# Autodesk Inventor assembly: Hanging Cupboard for Hood
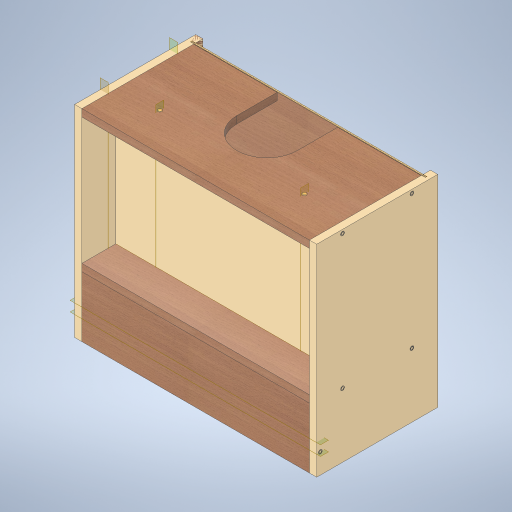
[picture p0: Inventor's stored thumbnail of the model, 512x512]
Saved by Autodesk Inventor 2024 (Build 280153000, 153)
## iProperties
RuleStatus: InUse
Created: 2017-01-20
Part Number: Hanging Cupboard for Hood
Document SubType Name: Assembly
Designer: SvetlanaB
Author: SvetlanaB
## Documents named in this file (12)
- C:\W4INV 2024 Design\iBOX LIBRARY\Kitchen\Wall Cabinets\Cupboard for Hood\Cupboard for Hood.iam
- C:\W4INV 2024 Design\iBOX LIBRARY\Kitchen\Wall Cabinets\Cupboard for Hood\Top panel.ipt
- C:\W4INV 2024 Design\iBOX LIBRARY\Kitchen\Wall Cabinets\Cupboard for Hood\Right panel.ipt
- C:\W4INV 2024 Design\iBOX LIBRARY\Kitchen\Wall Cabinets\Cupboard for Hood\Left panel.ipt
- C:\W4INV 2024 Design\iBOX LIBRARY\Kitchen\Wall Cabinets\Cupboard for Hood\Top panel2.ipt
- C:\W4INV 2024 Design\iBOX LIBRARY\Kitchen\Wall Cabinets\Cupboard for Hood\Bottom panel.ipt
- C:\W4INV 2024 Design\iBOX LIBRARY\Kitchen\Wall Cabinets\Cupboard for Hood\Back panel_1.ipt
- C:\W4INV 2024 Design\_LIBRARY\Fixed joints\Confirmat\CONFIRMAT\Confirmat L50 NB T18 PB T 18.ipt
- C:\W4INV 2024 Design\iBOX LIBRARY\Kitchen\Wall Cabinets\Cupboard for Hood\Hood cupboard concept.ipt
- C:\W4INV 2024 Design\iBOX LIBRARY\Kitchen\Wall Cabinets\Cupboard for Hood\Vertical partition.ipt
- C:\W4INV 2024 Design\_LIBRARY\Fixed joints\Confirmat\CONFIRMAT\Confirmat L50 & Cap D10 NB T18 PB T 18.ipt
- C:\W4INV 2023 Design\LIBRARY\Fixed joints\Confirmat\CONFIRMAT.ipt
## Components (22 placed, 10 different names)
1. @Skeleton
2. Top panel:1 — Pillar Board Side Plane:2, Pillar Board Side Plane:4, Pillar Board Side Plane:5, Pillar Board Side Plane:7, Nestled Board Plane:12, Nestled Board Plane:14, Flush:22
3. Right panel:1 — Nestled Board Plane:1, Nestled Board Plane:2, Nestled Board Plane:3, Nestled Board Plane:4, Nestled Board Plane:9
4. Left panel:1 — Flush:1, Flush:2, Nestled Board Plane:5, Nestled Board Plane:6, Nestled Board Plane:7, Nestled Board Plane:8, Nestled Board Plane:10, Mate:29, Mate:30
5. Top panel2:1 — Pillar Board Side Plane:1, Pillar Board Side Plane:3, Pillar Board Side Plane:6, Pillar Board Side Plane:8, Nestled Board Plane:11, Nestled Board Plane:13
6. Bottom panel:1 — Flush:5, Pillar Board Side Plane:9, Pillar Board Side Plane:10
7. Back panel_1:1 — Mate:29, Flush:22, Mate:30
8. Confirmat L50 NB T18 PB T 18:1 — Axis Plane:1, Pillar Board Side Plane:1, Nestled Board Plane:1
9. Confirmat L50 NB T18 PB T 18:2 — Axis Plane:2, Pillar Board Side Plane:2, Nestled Board Plane:2
10. Confirmat L50 NB T18 PB T 18:3 — Axis Plane:3, Pillar Board Side Plane:3, Nestled Board Plane:3
11. Confirmat L50 NB T18 PB T 18:4 — Axis Plane:4, Pillar Board Side Plane:4, Nestled Board Plane:4
12. Confirmat L50 NB T18 PB T 18:5 — Axis Plane:5, Pillar Board Side Plane:5, Nestled Board Plane:5
13. Confirmat L50 NB T18 PB T 18:6 — Axis Plane:6, Pillar Board Side Plane:6, Nestled Board Plane:6
14. Confirmat L50 NB T18 PB T 18:7 — Axis Plane:7, Pillar Board Side Plane:7, Nestled Board Plane:7
15. Confirmat L50 NB T18 PB T 18:8 — Axis Plane:8, Pillar Board Side Plane:8, Nestled Board Plane:8
16. Confirmat L50 NB T18 PB T 18:9 — Nestled Board Plane:9, Pillar Board Side Plane:9, Axis Plane:9
17. Confirmat L50 NB T18 PB T 18:10 — Nestled Board Plane:10, Pillar Board Side Plane:10, Axis Plane:10
18. Vertical partition:1 — Flush:16, Flush:17, Pillar Board Side Plane:11, Pillar Board Side Plane:12, Pillar Board Side Plane:13, Pillar Board Side Plane:14
19. Confirmat L50 & Cap D10 NB T18 PB T 18:11 — Axis Plane:11, Nestled Board Plane:11, Pillar Board Side Plane:11
20. Confirmat L50 & Cap D10 NB T18 PB T 18:12 — Axis Plane:12, Nestled Board Plane:12, Pillar Board Side Plane:12
21. Confirmat L50 & Cap D10 NB T18 PB T 18:13 — Axis Plane:13, Nestled Board Plane:13, Pillar Board Side Plane:13
22. Confirmat L50 & Cap D10 NB T18 PB T 18:14 — Axis Plane:14, Nestled Board Plane:14, Pillar Board Side Plane:14
## Relationships (50: Mate 30, Flush 20)
- Flush:1 (-64 mm): Left panel:1
- Flush:2 (-64 mm): Left panel:1
- Flush:5 (-50 mm): Bottom panel:1
- Axis Plane:1 [Mate]: Confirmat L50 NB T18 PB T 18:1
- Pillar Board Side Plane:1 [Mate] (-9 mm): Top panel2:1 ↔ Confirmat L50 NB T18 PB T 18:1
- Nestled Board Plane:1 [Flush]: Right panel:1 ↔ Confirmat L50 NB T18 PB T 18:1
- Axis Plane:2 [Mate]: Confirmat L50 NB T18 PB T 18:2
- Pillar Board Side Plane:2 [Mate] (-9 mm): Top panel:1 ↔ Confirmat L50 NB T18 PB T 18:2
- Nestled Board Plane:2 [Flush]: Right panel:1 ↔ Confirmat L50 NB T18 PB T 18:2
- Axis Plane:3 [Mate]: Confirmat L50 NB T18 PB T 18:3
- Pillar Board Side Plane:3 [Mate] (-9 mm): Top panel2:1 ↔ Confirmat L50 NB T18 PB T 18:3
- Nestled Board Plane:3 [Flush]: Right panel:1 ↔ Confirmat L50 NB T18 PB T 18:3
- Axis Plane:4 [Mate]: Confirmat L50 NB T18 PB T 18:4
- Pillar Board Side Plane:4 [Mate] (-9 mm): Top panel:1 ↔ Confirmat L50 NB T18 PB T 18:4
- Nestled Board Plane:4 [Flush]: Right panel:1 ↔ Confirmat L50 NB T18 PB T 18:4
- Axis Plane:5 [Mate]: Confirmat L50 NB T18 PB T 18:5
- Pillar Board Side Plane:5 [Mate] (-9 mm): Top panel:1 ↔ Confirmat L50 NB T18 PB T 18:5
- Nestled Board Plane:5 [Flush]: Left panel:1 ↔ Confirmat L50 NB T18 PB T 18:5
- Axis Plane:6 [Mate]: Confirmat L50 NB T18 PB T 18:6
- Pillar Board Side Plane:6 [Mate] (-9 mm): Top panel2:1 ↔ Confirmat L50 NB T18 PB T 18:6
- Nestled Board Plane:6 [Flush]: Left panel:1 ↔ Confirmat L50 NB T18 PB T 18:6
- Axis Plane:7 [Mate]: Confirmat L50 NB T18 PB T 18:7
- Pillar Board Side Plane:7 [Mate] (-9 mm): Top panel:1 ↔ Confirmat L50 NB T18 PB T 18:7
- Nestled Board Plane:7 [Flush]: Left panel:1 ↔ Confirmat L50 NB T18 PB T 18:7
- Axis Plane:8 [Mate]: Confirmat L50 NB T18 PB T 18:8
- Pillar Board Side Plane:8 [Mate] (-9 mm): Top panel2:1 ↔ Confirmat L50 NB T18 PB T 18:8
- Nestled Board Plane:8 [Flush]: Left panel:1 ↔ Confirmat L50 NB T18 PB T 18:8
- Nestled Board Plane:9 [Flush]: Right panel:1 ↔ Confirmat L50 NB T18 PB T 18:9
- Pillar Board Side Plane:9 [Mate] (-9 mm): Bottom panel:1 ↔ Confirmat L50 NB T18 PB T 18:9
- Axis Plane:9 [Mate]: Confirmat L50 NB T18 PB T 18:9
- Nestled Board Plane:10 [Flush]: Left panel:1 ↔ Confirmat L50 NB T18 PB T 18:10
- Pillar Board Side Plane:10 [Mate] (-9 mm): Bottom panel:1 ↔ Confirmat L50 NB T18 PB T 18:10
- Axis Plane:10 [Mate]: Confirmat L50 NB T18 PB T 18:10
- Flush:16 (-100 mm): Vertical partition:1
- Flush:17 (-100 mm): Vertical partition:1
- Axis Plane:11 [Mate]: Confirmat L50 & Cap D10 NB T18 PB T 18:11
- Nestled Board Plane:11 [Flush]: Top panel2:1 ↔ Confirmat L50 & Cap D10 NB T18 PB T 18:11
- Pillar Board Side Plane:11 [Mate] (-9 mm): Vertical partition:1 ↔ Confirmat L50 & Cap D10 NB T18 PB T 18:11
- Axis Plane:12 [Mate]: Confirmat L50 & Cap D10 NB T18 PB T 18:12
- Nestled Board Plane:12 [Flush]: Top panel:1 ↔ Confirmat L50 & Cap D10 NB T18 PB T 18:12
- Pillar Board Side Plane:12 [Mate] (-9 mm): Vertical partition:1 ↔ Confirmat L50 & Cap D10 NB T18 PB T 18:12
- Axis Plane:13 [Mate]: Confirmat L50 & Cap D10 NB T18 PB T 18:13
- Nestled Board Plane:13 [Flush]: Top panel2:1 ↔ Confirmat L50 & Cap D10 NB T18 PB T 18:13
- Pillar Board Side Plane:13 [Mate] (-9 mm): Vertical partition:1 ↔ Confirmat L50 & Cap D10 NB T18 PB T 18:13
- Axis Plane:14 [Mate]: Confirmat L50 & Cap D10 NB T18 PB T 18:14
- Nestled Board Plane:14 [Flush]: Top panel:1 ↔ Confirmat L50 & Cap D10 NB T18 PB T 18:14
- Pillar Board Side Plane:14 [Mate] (-9 mm): Vertical partition:1 ↔ Confirmat L50 & Cap D10 NB T18 PB T 18:14
- Mate:29: Left panel:1 ↔ Back panel_1:1
- Flush:22: Top panel:1 ↔ Back panel_1:1
- Mate:30 (0.5 mm): Left panel:1 ↔ Back panel_1:1
## Named parameters: Panel_thickness = 18 mm
